# Autodesk Inventor assembly: 0008-10-10 Injectomat Standard_Seringa 20
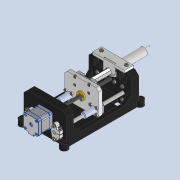
[picture p0: Inventor's stored thumbnail of the model, 180x180]
Saved by Autodesk Inventor 2020 (Build 240168000, 168)
## iProperties
Created: 2021-02-20
Part Number: 0008-10-10 Injectomat Standard_Seringa 20
Document SubType Name: Assembly
Designer: Iulian Bors
Mass: 1274.49 g
Surface Area: 2683.15 cm^2
Volume: 830.675 cm^3
Density: 1.53428 g/cm^3
Description: Injectomat standard
Author: Iulian Bors
Subject: 10-10
## Documents named in this file (28)
- Z:\I.A.B\Proiecte\0008 I.A.B 3D 2.1 Imprimanta aracet Metal\10 Mecanic\0008-10-10 Injectomat Standard_Seringa 20.iam
- Z:\I.A.B\Proiecte\0008 I.A.B 3D 2.1 Imprimanta aracet Metal\10 Mecanic\0008-10-1000 LMK8LUU.ipt
- Z:\I.A.B\Proiecte\0008 I.A.B 3D 2.1 Imprimanta aracet Metal\10 Mecanic\0008-10-1002  Hub.ipt
- Z:\I.A.B\Proiecte\0008 I.A.B 3D 2.1 Imprimanta aracet Metal\10 Mecanic\0008-10-1001 NEMA17 - Motor de passo.ipt
- Z:\I.A.B\Proiecte\0008 I.A.B 3D 2.1 Imprimanta aracet Metal\10 Mecanic\0008-10-1003 T8 screw.ipt
- Z:\I.A.B\Proiecte\0008 I.A.B 3D 2.1 Imprimanta aracet Metal\10 Mecanic\0008-10-001.ipt
- Z:\I.A.B\Proiecte\0008 I.A.B 3D 2.1 Imprimanta aracet Metal\10 Mecanic\0008-10-1005 ISO 1224-1 - 10 - 8 x 22 x 7.ipt
- Z:\I.A.B\Proiecte\0008 I.A.B 3D 2.1 Imprimanta aracet Metal\10 Mecanic\0008-10-002 Corp_Injectomat1.ipt
- Z:\I.A.B\Proiecte\0008 I.A.B 3D 2.1 Imprimanta aracet Metal\10 Mecanic\0008-10-1004 Piulita.ipt
- Z:\I.A.B\Proiecte\0008 I.A.B 3D 2.1 Imprimanta aracet Metal\10 Mecanic\0008-10-003.ipt
- Z:\I.A.B\Proiecte\0008 I.A.B 3D 2.1 Imprimanta aracet Metal\10 Mecanic\0008-10-1006 SHF8.ipt
- Z:\I.A.B\Proiecte\0008 I.A.B 3D 2.1 Imprimanta aracet Metal\10 Mecanic\0008-10-1007 Bara 8.ipt
- Z:\I.A.B\Proiecte\0008 I.A.B 3D 2.1 Imprimanta aracet Metal\10 Mecanic\SurubM4x25.iam
- Z:\I.A.B\Proiecte\0008 I.A.B 3D 2.1 Imprimanta aracet Metal\10 Mecanic\SurubM4x35.iam
- Z:\I.A.B\Proiecte\0008 I.A.B 3D 2.1 Imprimanta aracet Metal\10 Mecanic\m3X16.iam
- Z:\I.A.B\Proiecte\0008 I.A.B 3D 2.1 Imprimanta aracet Metal\10 Mecanic\0008-10-2006 DIN 7984 - M3 x 16.ipt
- Z:\I.A.B\Proiecte\0008 I.A.B 3D 2.1 Imprimanta aracet Metal\10 Mecanic\0008-10-2007 DIN 7984 - M4 x 16.ipt
- Z:\I.A.B\Proiecte\0008 I.A.B 3D 2.1 Imprimanta aracet Metal\10 Mecanic\0008-10-2001 DIN 934 - M4 x 0.7.ipt
- Z:\I.A.B\Proiecte\0008 I.A.B 3D 2.1 Imprimanta aracet Metal\10 Mecanic\0008-10-005 Suport_Rulment.ipt
- Z:\I.A.B\Proiecte\0008 I.A.B 3D 2.1 Imprimanta aracet Metal\10 Mecanic\0008-10-2000 DIN 6912 - M4 x 25.ipt
- Z:\I.A.B\Proiecte\0008 I.A.B 3D 2.1 Imprimanta aracet Metal\10 Mecanic\0008-10-2008 DIN 912 - M3 x 0.5 x 25 x 18.ipt
- Z:\I.A.B\Proiecte\0008 I.A.B 3D 2.1 Imprimanta aracet Metal\10 Mecanic\0008-10-2005 DIN 125 - A 3.2.ipt
- Z:\I.A.B\Proiecte\0008 I.A.B 3D 2.1 Imprimanta aracet Metal\10 Mecanic\0008-10-2009 DIN 555-5 - M3.ipt
- Z:\I.A.B\Proiecte\0008 I.A.B 3D 2.1 Imprimanta aracet Metal\10 Mecanic\Seringa\Seringa 20 Ml\body 20ml_Défaut.ipt
- Z:\I.A.B\Proiecte\0008 I.A.B 3D 2.1 Imprimanta aracet Metal\10 Mecanic\Seringa\Seringa 20 Ml\plunger_Défaut.ipt
- Z:\I.A.B\Proiecte\0008 I.A.B 3D 2.1 Imprimanta aracet Metal\10 Mecanic\Seringa\Seringa 20 Ml\rubber plunger_Défaut.ipt
- Z:\I.A.B\Proiecte\0008 I.A.B 3D 2.1 Imprimanta aracet Metal\10 Mecanic\0008-10-057  Fixare seringa 20 Ml.ipt
- Z:\I.A.B\Proiecte\0008 I.A.B 3D 2.1 Imprimanta aracet Metal\10 Mecanic\0008-10-058.ipt
## Components (76 placed, 29 different names)
1. 0008-10-1000 LMK8LUU.ipt:4 — Insert:6, Angle:5, Mate:13, Mate:17
2. 0008-10-1000 LMK8LUU.ipt:5 — Insert:5, Angle:4, Mate:12, Mate:15, Insert:30
3. 0008-10-1002  Hub.ipt:6 — Insert:2, Insert:3
4. 0008-10-1001 NEMA17 - Motor de passo.ipt:7 — Insert:3, Angle:2, Mate:5
5. 0008-10-1003 T8 screw.ipt:8 — Insert:2, Mate:21
6. 0008-10-001.ipt:9 — Angle:3, Flush:3, Insert:5, Angle:4, Insert:6, Angle:5, Mate:6, Mate:7, Insert:7, Mate:8, Mate:9, Mate:10, Tangent:2
7. 0008-10-002 Corp_Injectomat1.ipt:10 — Mate:5, Mate:6, Mate:7, Mate:11, Mate:14, Mate:16, Mate:18, Angle:7, Angle:9, Insert:32, Insert:44, Insert:48, Insert:49, Insert:50, Mate:24, Flush:6, Tangent:1, Angle:12
8. 0008-10-1004 Piulita.ipt:11 — Insert:7, Insert:28, Mate:21
9. 0008-10-003.ipt:12 — Mate:8, Mate:9, Mate:10, Insert:23, Insert:24, Insert:25, Insert:26, Flush:5, Mate:26, Mate:27, Flush:7
10. 0008-10-1006 SHF8.ipt:13 — Mate:11, Mate:12, Insert:8, Angle:9, Insert:15, Insert:16, Insert:36
11. 0008-10-1007 Bara 8.ipt:14 — Insert:8
12. 0008-10-1007 Bara 8.ipt:15 — Insert:9
13. 0008-10-1006 SHF8.ipt:16 — Mate:13, Mate:14, Insert:9, Angle:10, Insert:17, Insert:18, Insert:38
14. 0008-10-1006 SHF8.ipt:17 — Mate:15, Mate:16, Angle:8, Insert:19, Insert:20, Insert:41
15. 0008-10-1006 SHF8.ipt:18 — Mate:17, Mate:18, Angle:7, Insert:21, Insert:22, Insert:42
16. 0008-10-004 Fixare seringa.ipt:19 — Insert:10, Insert:11, Flush:6
17. SurubM4x25.iam:20 [sub-assembly] — Insert:10
18. SurubM4x25.iam:21 [sub-assembly] — Insert:11
19. SurubM4x35.iam:22 [sub-assembly] — Insert:15
20. SurubM4x35.iam:23 [sub-assembly] — Insert:16
21. SurubM4x35.iam:24 [sub-assembly] — Insert:18
22. SurubM4x35.iam:25 [sub-assembly] — Insert:17
23. SurubM4x35.iam:26 [sub-assembly] — Insert:21
24. SurubM4x35.iam:27 [sub-assembly] — Insert:22
25. SurubM4x35.iam:28 [sub-assembly] — Insert:19
26. SurubM4x35.iam:29 [sub-assembly] — Insert:20
27. m3X16.iam:30 [sub-assembly] — Insert:23
28. m3X16.iam:31 [sub-assembly] — Insert:24
29. m3X16.iam:32 [sub-assembly] — Insert:25
30. m3X16.iam:33 [sub-assembly] — Insert:26
31. 0008-10-005 Suport_Rulment.ipt:58 — Insert:31, Angle:11, Insert:33, Insert:34
32. 0008-10-1005 ISO 1224-1 - 10 - 8 x 22 x 7.ipt:59 — Insert:31, Insert:32
33. SurubM4x35.iam:60 [sub-assembly] — Insert:34
34. SurubM4x35.iam:61 [sub-assembly] — Insert:33
35. 0008-10-2001 DIN 934 - M4 x 0.7.ipt:62 — Insert:35
36. 0008-10-2000 DIN 6912 - M4 x 25.ipt:63 — Insert:35, Insert:36
37. 0008-10-2001 DIN 934 - M4 x 0.7.ipt:64
38. 0008-10-2000 DIN 6912 - M4 x 25.ipt:65 — Insert:38
39. 0008-10-2001 DIN 934 - M4 x 0.7.ipt:66
40. 0008-10-2000 DIN 6912 - M4 x 25.ipt:67 — Insert:41
41. 0008-10-2001 DIN 934 - M4 x 0.7.ipt:68
42. 0008-10-2000 DIN 6912 - M4 x 25.ipt:69 — Insert:42
43. 0008-10-2008 DIN 912 - M3 x 0.5 x 25 x 18.ipt:70 — Insert:43
44. 0008-10-2005 DIN 125 - A 3.2.ipt:71 — Insert:43, Insert:44
45. 0008-10-2008 DIN 912 - M3 x 0.5 x 25 x 18.ipt:72
46. 0008-10-2005 DIN 125 - A 3.2.ipt:73 — Insert:50
47. 0008-10-2008 DIN 912 - M3 x 0.5 x 25 x 18.ipt:74
48. 0008-10-2005 DIN 125 - A 3.2.ipt:75 — Insert:48
49. 0008-10-2008 DIN 912 - M3 x 0.5 x 25 x 18.ipt:76
50. 0008-10-2005 DIN 125 - A 3.2.ipt:77 — Insert:49
51. body 20ml_Défaut:1 — Mate:22, Tangent:1, Angle:12
52. plunger_Défaut:1 — Insert:51, Mate:24, Flush:5, Tangent:2
53. rubber plunger_Défaut:1 — Insert:51, Mate:22
54. 0008-10-058:1 — Mate:26, Mate:27, Flush:7
55. 0008-10-2006 DIN 7984 - M3 x 16.ipt:34 — Insert:27, Insert:28
56. 0008-10-2009 DIN 555-5 - M3.ipt:35 — Insert:27
57. DIN 7984 M3 x 16:2
58. DIN 555 - replaced by DIN EN 24034 M3:6
59. DIN 7984 M3 x 16:3
60. DIN 555 - replaced by DIN EN 24034 M3:7
61. 0008-10-2001 DIN 934 - M4 x 0.7.ipt:42 — Insert:29
62. 0008-10-2007 DIN 7984 - M4 x 16.ipt:43 — Insert:29, Insert:30
63. 0008-10-2001 DIN 934 - M4 x 0.7.ipt:44
64. 0008-10-2007 DIN 7984 - M4 x 16.ipt:45
65. 0008-10-2001 DIN 934 - M4 x 0.7.ipt:46
66. 0008-10-2007 DIN 7984 - M4 x 16.ipt:47
67. 0008-10-2001 DIN 934 - M4 x 0.7.ipt:48
68. 0008-10-2007 DIN 7984 - M4 x 16.ipt:49
69. 0008-10-2001 DIN 934 - M4 x 0.7.ipt:50
70. 0008-10-2007 DIN 7984 - M4 x 16.ipt:51
71. 0008-10-2001 DIN 934 - M4 x 0.7.ipt:52
72. 0008-10-2007 DIN 7984 - M4 x 16.ipt:53
73. 0008-10-2001 DIN 934 - M4 x 0.7.ipt:54
74. 0008-10-2007 DIN 7984 - M4 x 16.ipt:55
75. 0008-10-2001 DIN 934 - M4 x 0.7.ipt:56
76. 0008-10-2007 DIN 7984 - M4 x 16.ipt:57
## Component patterns: (2 elements), (3 elements, first: 0008-10-2006 DIN 7984 - M3 x 16.ipt:34 + 0008-10-2009 DIN 555-5 - M3.ipt:35), (4 elements, first: 0008-10-2001 DIN 934 - M4 x 0.7.ipt:42 + 0008-10-2007 DIN 7984 - M4 x 16.ipt:43), Component Pattern 2:2 (4 elements)
## Relationships (81: Insert 46, Mate 19, Angle 10, Flush 4, Tangent 2)
- Insert:2: 0008-10-1002  Hub.ipt:6 ↔ 0008-10-1003 T8 screw.ipt:8
- Insert:3: 0008-10-1002  Hub.ipt:6 ↔ 0008-10-1001 NEMA17 - Motor de passo.ipt:7
- Angle:2 (0 deg): 0008-10-1001 NEMA17 - Motor de passo.ipt:7
- Angle:3 (0 deg): 0008-10-001.ipt:9
- Flush:3 (-13.343 mm): 0008-10-001.ipt:9
- Insert:5: 0008-10-1000 LMK8LUU.ipt:5 ↔ 0008-10-001.ipt:9
- Angle:4 (0 deg): 0008-10-1000 LMK8LUU.ipt:5 ↔ 0008-10-001.ipt:9
- Insert:6: 0008-10-1000 LMK8LUU.ipt:4 ↔ 0008-10-001.ipt:9
- Angle:5 (0 deg): 0008-10-1000 LMK8LUU.ipt:4 ↔ 0008-10-001.ipt:9
- Mate:5: 0008-10-1001 NEMA17 - Motor de passo.ipt:7 ↔ 0008-10-002 Corp_Injectomat1.ipt:10
- Mate:6: 0008-10-001.ipt:9 ↔ 0008-10-002 Corp_Injectomat1.ipt:10
- Mate:7 (5 mm): 0008-10-001.ipt:9 ↔ 0008-10-002 Corp_Injectomat1.ipt:10
- Insert:7: 0008-10-001.ipt:9 ↔ 0008-10-1004 Piulita.ipt:11
- Mate:8: 0008-10-001.ipt:9 ↔ 0008-10-003.ipt:12
- Mate:9 (-27 mm): 0008-10-001.ipt:9 ↔ 0008-10-003.ipt:12
- Mate:10: 0008-10-001.ipt:9 ↔ 0008-10-003.ipt:12
- Mate:11: 0008-10-002 Corp_Injectomat1.ipt:10 ↔ 0008-10-1006 SHF8.ipt:13
- Mate:12: 0008-10-1000 LMK8LUU.ipt:5 ↔ 0008-10-1006 SHF8.ipt:13
- Insert:8: 0008-10-1006 SHF8.ipt:13 ↔ 0008-10-1007 Bara 8.ipt:14
- Mate:13: 0008-10-1000 LMK8LUU.ipt:4 ↔ 0008-10-1006 SHF8.ipt:16
- Mate:14: 0008-10-002 Corp_Injectomat1.ipt:10 ↔ 0008-10-1006 SHF8.ipt:16
- Mate:15: 0008-10-1000 LMK8LUU.ipt:5 ↔ 0008-10-1006 SHF8.ipt:17
- Mate:16: 0008-10-002 Corp_Injectomat1.ipt:10 ↔ 0008-10-1006 SHF8.ipt:17
- Mate:17: 0008-10-1000 LMK8LUU.ipt:4 ↔ 0008-10-1006 SHF8.ipt:18
- Mate:18: 0008-10-002 Corp_Injectomat1.ipt:10 ↔ 0008-10-1006 SHF8.ipt:18
- Insert:9: 0008-10-1007 Bara 8.ipt:15 ↔ 0008-10-1006 SHF8.ipt:16
- Angle:7 (0 deg): 0008-10-002 Corp_Injectomat1.ipt:10 ↔ 0008-10-1006 SHF8.ipt:18
- Angle:8 (180 deg): 0008-10-1006 SHF8.ipt:17
- Angle:9 (0 deg): 0008-10-002 Corp_Injectomat1.ipt:10 ↔ 0008-10-1006 SHF8.ipt:13
- Angle:10 (0 deg): 0008-10-1006 SHF8.ipt:16
- Insert:10: 0008-10-004 Fixare seringa.ipt:19 ↔ SurubM4x25.iam:20
- Insert:11: 0008-10-004 Fixare seringa.ipt:19 ↔ SurubM4x25.iam:21
- Insert:15: 0008-10-1006 SHF8.ipt:13 ↔ SurubM4x35.iam:22
- Insert:16: 0008-10-1006 SHF8.ipt:13 ↔ SurubM4x35.iam:23
- Insert:17: 0008-10-1006 SHF8.ipt:16 ↔ SurubM4x35.iam:25
- Insert:18: 0008-10-1006 SHF8.ipt:16 ↔ SurubM4x35.iam:24
- Insert:19: 0008-10-1006 SHF8.ipt:17 ↔ SurubM4x35.iam:28
- Insert:20: 0008-10-1006 SHF8.ipt:17 ↔ SurubM4x35.iam:29
- Insert:21: 0008-10-1006 SHF8.ipt:18 ↔ SurubM4x35.iam:26
- Insert:22: 0008-10-1006 SHF8.ipt:18 ↔ SurubM4x35.iam:27
- Insert:23: 0008-10-003.ipt:12 ↔ m3X16.iam:30
- Insert:24: 0008-10-003.ipt:12 ↔ m3X16.iam:31
- Insert:25: 0008-10-003.ipt:12 ↔ m3X16.iam:32
- Insert:26: 0008-10-003.ipt:12 ↔ m3X16.iam:33
- Insert:27: 0008-10-2006 DIN 7984 - M3 x 16.ipt:34 ↔ 0008-10-2009 DIN 555-5 - M3.ipt:35
- Insert:28: 0008-10-1004 Piulita.ipt:11 ↔ 0008-10-2006 DIN 7984 - M3 x 16.ipt:34
- Insert:29: 0008-10-2001 DIN 934 - M4 x 0.7.ipt:42 ↔ 0008-10-2007 DIN 7984 - M4 x 16.ipt:43
- Insert:30: 0008-10-1000 LMK8LUU.ipt:5 ↔ 0008-10-2007 DIN 7984 - M4 x 16.ipt:43
- Mate:21: 0008-10-1003 T8 screw.ipt:8 ↔ 0008-10-1004 Piulita.ipt:11
- Insert:31: 0008-10-005 Suport_Rulment.ipt:58 ↔ 0008-10-1005 ISO 1224-1 - 10 - 8 x 22 x 7.ipt:59
- Insert:32: 0008-10-002 Corp_Injectomat1.ipt:10 ↔ 0008-10-1005 ISO 1224-1 - 10 - 8 x 22 x 7.ipt:59
- Angle:11 (0 deg): 0008-10-005 Suport_Rulment.ipt:58
- Insert:33: 0008-10-005 Suport_Rulment.ipt:58 ↔ SurubM4x35.iam:61
- Insert:34: 0008-10-005 Suport_Rulment.ipt:58 ↔ SurubM4x35.iam:60
- Insert:35: 0008-10-2001 DIN 934 - M4 x 0.7.ipt:62 ↔ 0008-10-2000 DIN 6912 - M4 x 25.ipt:63
- Insert:36: 0008-10-1006 SHF8.ipt:13 ↔ 0008-10-2000 DIN 6912 - M4 x 25.ipt:63
- [Insert]: 0008-10-2001 DIN 934 - M4 x 0.7.ipt:64 ↔ 0008-10-2000 DIN 6912 - M4 x 25.ipt:65
- Insert:38: 0008-10-1006 SHF8.ipt:16 ↔ 0008-10-2000 DIN 6912 - M4 x 25.ipt:65
- [Insert]: 0008-10-2001 DIN 934 - M4 x 0.7.ipt:66 ↔ 0008-10-2000 DIN 6912 - M4 x 25.ipt:67
- [Insert]: 0008-10-2001 DIN 934 - M4 x 0.7.ipt:68 ↔ 0008-10-2000 DIN 6912 - M4 x 25.ipt:69
- Insert:41: 0008-10-1006 SHF8.ipt:17 ↔ 0008-10-2000 DIN 6912 - M4 x 25.ipt:67
- Insert:42: 0008-10-1006 SHF8.ipt:18 ↔ 0008-10-2000 DIN 6912 - M4 x 25.ipt:69
- Insert:43: 0008-10-2008 DIN 912 - M3 x 0.5 x 25 x 18.ipt:70 ↔ 0008-10-2005 DIN 125 - A 3.2.ipt:71
- Insert:44: 0008-10-002 Corp_Injectomat1.ipt:10 ↔ 0008-10-2005 DIN 125 - A 3.2.ipt:71
- [Insert]: 0008-10-2008 DIN 912 - M3 x 0.5 x 25 x 18.ipt:72 ↔ 0008-10-2005 DIN 125 - A 3.2.ipt:73
- [Insert]: 0008-10-2008 DIN 912 - M3 x 0.5 x 25 x 18.ipt:74 ↔ 0008-10-2005 DIN 125 - A 3.2.ipt:75
- [Insert]: 0008-10-2008 DIN 912 - M3 x 0.5 x 25 x 18.ipt:76 ↔ 0008-10-2005 DIN 125 - A 3.2.ipt:77
- Insert:48: 0008-10-002 Corp_Injectomat1.ipt:10 ↔ 0008-10-2005 DIN 125 - A 3.2.ipt:75
- Insert:49: 0008-10-002 Corp_Injectomat1.ipt:10 ↔ 0008-10-2005 DIN 125 - A 3.2.ipt:77
- Insert:50: 0008-10-002 Corp_Injectomat1.ipt:10 ↔ 0008-10-2005 DIN 125 - A 3.2.ipt:73
- Insert:51: plunger_Défaut:1 ↔ rubber plunger_Défaut:1
- Mate:22: body 20ml_Défaut:1 ↔ rubber plunger_Défaut:1
- Mate:24: 0008-10-002 Corp_Injectomat1.ipt:10 ↔ plunger_Défaut:1
- Flush:5 (18.184 mm): 0008-10-003.ipt:12 ↔ plunger_Défaut:1
- Flush:6: 0008-10-002 Corp_Injectomat1.ipt:10 ↔ 0008-10-004 Fixare seringa.ipt:19
- Tangent:1: 0008-10-002 Corp_Injectomat1.ipt:10 ↔ body 20ml_Défaut:1
- Angle:12 (180 deg): 0008-10-002 Corp_Injectomat1.ipt:10 ↔ body 20ml_Défaut:1
- Tangent:2: 0008-10-001.ipt:9 ↔ plunger_Défaut:1
- Mate:26: 0008-10-003.ipt:12 ↔ 0008-10-058:1
- Mate:27 (0.5 mm): 0008-10-003.ipt:12 ↔ 0008-10-058:1
- Flush:7: 0008-10-003.ipt:12 ↔ 0008-10-058:1
## Named parameters: d90_d88 = 0 mm, d92_d88 = 0 mm, d93_d88 = 0 mm, d98_d96 = 0 mm, d99_d96 = 0 mm, d100_d96 = 0 mm
